# Autodesk Inventor assembly: 組合1
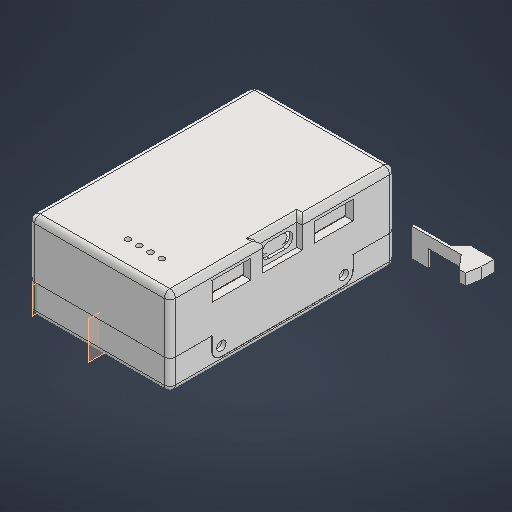
[picture p0: Inventor's stored thumbnail of the model, 512x512]
Saved by Autodesk Inventor 2026.2 (Build 302298010, 298A)
## iProperties
Created: 2026-03-29
Part Number: 組合1
Document SubType Name: Assembly
Designer: gavin
Author: gavin
## Documents named in this file (6)
- D:\Inventor\power bank v1.1 mini\組合1.iam
- D:\Inventor\power bank v1.1 mini\18650 budge head.ipt
- D:\Inventor\power bank v1.1 mini\circuit board.ipt
- D:\Inventor\power bank v1.1 mini\buttom case.ipt
- D:\Inventor\power bank v1.1 mini\top case.ipt
- D:\Inventor\power bank v1.1 mini\botton.ipt
## Components (5 placed, 5 different names)
1. circuit board:1 — 貼合:4, 貼合:5, 貼合:6
2. 18650 budge head:5 — 貼合:1, 相切:5, 貼合:2
3. buttom case:1 — 貼合:1, 相切:5, 貼合:2, 齊平:5, 齊平:6, 貼合:3
4. top case:1 — 齊平:5, 齊平:6, 貼合:3, 貼合:4, 貼合:5, 貼合:6
5. botton:1
## Relationships (9: Mate 6, Flush 2, Tangent 1)
- 貼合:1 [Mate]: 18650 budge head:5 ↔ buttom case:1
- 相切:5 [Tangent]: 18650 budge head:5 ↔ buttom case:1
- 貼合:2 [Mate]: 18650 budge head:5 ↔ buttom case:1
- 齊平:5 [Flush]: buttom case:1 ↔ top case:1
- 齊平:6 [Flush]: buttom case:1 ↔ top case:1
- 貼合:3 [Mate]: buttom case:1 ↔ top case:1
- 貼合:4 [Mate] (-1.5 mm): circuit board:1 ↔ top case:1
- 貼合:5 [Mate] (0.1 mm): circuit board:1 ↔ top case:1
- 貼合:6 [Mate] (0.38 mm): circuit board:1 ↔ top case:1
